# Autodesk Inventor assembly: VER2.0_MIR_CPY_MIR1
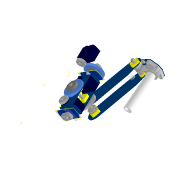
[picture p0: Inventor's stored thumbnail of the model, 180x180]
Saved by Autodesk Inventor 2020.5 (Build 245400000, 400)
## iProperties
Created: 2022-10-31
Part Number: VER2.0_MIR_CPY_MIR1
Document SubType Name: Assembly
Designer: Administrator
Author: Administrator
## Documents named in this file (17)
- C:\Users\Administrator\Documents\kamuy2\kamuy2\VER2.0_MIR_CPY_MIR1.iam
- C:\Users\Administrator\Documents\kamuy2\kamuy2\Parts\Part2_MIR_CPY_MIR1.ipt
- C:\Users\Administrator\Documents\kamuy2\kamuy2\Parts\x-540_idle_MIR_CPY_MIR1.ipt
- C:\Users\Administrator\Documents\kamuy2\kamuy2\Parts\GEABP1.0-32-10-A-12-KFC22-K3_Autodesk_Inventor_2020_20221101\AIS2020\GEABP1_0-32-10-A-12-KFC22-K3_MIR_CPY_MIR1.iam
- C:\Users\Administrator\Documents\kamuy2\kamuy2\Parts\GEYK1.0-70-10-B-10K_Autodesk_Inventor_2020_20221114\AIS2020\GEYK1_0-70-10-B-10K_MIR_CPY_MIR1.iam
- C:\Users\Administrator\Documents\kamuy2\kamuy2\Part16_MIR_CPY_MIR1.ipt
- C:\Users\Administrator\Documents\kamuy2\kamuy2\Part1_MIR_CPY_MIR1.ipt
- C:\Users\Administrator\Documents\kamuy2\kamuy2\Part13_MIR_CPY_MIR1.ipt
- C:\Users\Administrator\Documents\kamuy2\kamuy2\Part17_MIR_CPY_MIR1.ipt
- C:\Users\Administrator\Documents\kamuy2\kamuy2\Parts\SMYHF10_STEP_AP203AP214\SMYHF10_203_MIR_CPY_MIR1.ipt
- C:\Users\Administrator\Documents\kamuy2\kamuy2\Parts\BGHK6800VV-30_Autodesk_Inventor_2020_20221102\AIS2020\BGHK6800VV-30_MIR_CPY_MIR1.iam
- C:\Users\Administrator\Documents\kamuy2\kamuy2\Parts\XW540.N105.I101_MIR_CPY_MIR1.ipt
- C:\Users\Administrator\Documents\kamuy2\kamuy2\Parts\NSFMKR10-67-KA22-A20_Autodesk_Inventor_2020_20221116\AIS2020\NSFMKR10-67-KA22-A20_MIR_CPY_MIR1.iam
- C:\Users\Administrator\Documents\kamuy2\kamuy2\Parts\NSFMR10-37_Autodesk_Inventor_2020_20221116\AIS2020\NSFMR10-37(000_000)_MIR_CPY_MIR1.iam
- C:\Users\Administrator\Documents\kamuy2\kamuy2\Parts\NSFMKRRA10-144-F3-S6-KA5-A18-KB108.5-B11_Autodesk_Inventor_2020_20221117\AIS2020\NSFMKRRA10-144-F3-S6-KA5-A18-KB108_5-B11_MIR_CPY_MIR1.iam
- C:\Users\Administrator\Documents\kamuy2\kamuy2\LEG_MIR_MIR2.iam
- C:\Users\Administrator\Documents\kamuy2\kamuy2\Parts\BGTAB6900VV_Autodesk_Inventor_2020_20221121\AIS2020\BGTAB6900VV_MIR.iam
## Components (26 placed, 16 different names)
1. Part2_MIR_CPY_MIR1:1
2. x-540_idle_MIR_CPY_MIR1:1 — メイト:51, メイト:50, フラッシュ:68, フラッシュ:66, フラッシュ:58, メイト:258, メイト:154, メイト:166, フラッシュ:103, メイト:256
3. GEABP1_0-32-10-A-12-KFC22-K3_MIR_CPY_MIR1:1 [sub-assembly] — メイト:51, メイト:50, フラッシュ:31
4. GEYK1_0-70-10-B-10K_MIR_CPY_MIR1:1 [sub-assembly] — フラッシュ:61, フラッシュ:136, メイト:248
5. x-540_idle_MIR_CPY_MIR1:2 — フラッシュ:68, フラッシュ:66, フラッシュ:58, メイト:86, メイト:85, メイト:168, フラッシュ:100, メイト:183, メイト:180, メイト:179, メイト:178
6. GEABP1_0-32-10-A-12-KFC22-K3_MIR_CPY_MIR1:2 [sub-assembly] — フラッシュ:61, メイト:86, メイト:85
7. Part16_MIR_CPY_MIR1:1 — メイト:258, フラッシュ:92, メイト:170
8. Part16_MIR_CPY_MIR1:2 — メイト:168, メイト:154, フラッシュ:92, メイト:66, フラッシュ:141, メイト:67
9. Part1_MIR_CPY_MIR1:1 — メイト:66, フラッシュ:141, フラッシュ:100
10. Part1_MIR_CPY_MIR1:2 — メイト:183, メイト:170, メイト:166
11. Part13_MIR_CPY_MIR1:1 — フラッシュ:103, フラッシュ:108, フラッシュ:104, メイト:172, メイト:208
12. Part17_MIR_CPY_MIR1:1 — フラッシュ:108, フラッシュ:104, メイト:172, フラッシュ:105, メイト:174, メイト:177
13. SMYHF10_203_MIR_CPY_MIR1:1 — フラッシュ:105, メイト:174, メイト:254
14. GEYK1_0-70-10-B-10K_MIR_CPY_MIR1:2 [sub-assembly] — メイト:177, メイト:207, メイト:42
15. Part13_MIR_CPY_MIR1:2 — メイト:180, メイト:179, メイト:178, フラッシュ:110, メイト:194, メイト:214
16. SMYHF10_203_MIR_CPY_MIR1:2 — メイト:187, メイト:185, メイト:213
17. Part17_MIR_CPY_MIR1:2 — フラッシュ:110, メイト:194, メイト:187, メイト:185, メイト:211, メイト:215, メイト:69
18. GEABP1_0-32-10-A-12-KFC22-K3_MIR_CPY_MIR1:3 [sub-assembly] — メイト:204, メイト:203
19. XW540.N105.I101_MIR_CPY_MIR1:1 — メイト:204, メイト:203, メイト:41
20. NSFMKR10-67-KA22-A20_MIR_CPY_MIR1:1 [sub-assembly] — メイト:254, メイト:208, メイト:207, メイト:40
21. BGHK6800VV-30_MIR_CPY_MIR1:2 [sub-assembly] — メイト:211, メイト:212
22. NSFMR10-37(000_000)_MIR_CPY_MIR1:1 [sub-assembly] — メイト:215, メイト:214, メイト:213, メイト:212, メイト:68
23. NSFMKRRA10-144-F3-S6-KA5-A18-KB108_5-B11_MIR_CPY_MIR1:1 [sub-assembly] — メイト:67, メイト:256, フラッシュ:136, メイト:248, メイト:64
24. LEG_MIR_MIR2:1 [sub-assembly] — フラッシュ:31, メイト:64
25. BGTAB6900VV_MIR:1 [sub-assembly] — メイト:69, メイト:68, フラッシュ:19
26. BGTAB6900VV_MIR:2 [sub-assembly] — メイト:40, メイト:41, メイト:42, フラッシュ:19
## Relationships (54: Mate 39, Flush 15)
- メイト:51 [Mate]: x-540_idle_MIR_CPY_MIR1:1 ↔ GEABP1_0-32-10-A-12-KFC22-K3_MIR_CPY_MIR1:1
- メイト:50 [Mate] (4 mm): x-540_idle_MIR_CPY_MIR1:1 ↔ GEABP1_0-32-10-A-12-KFC22-K3_MIR_CPY_MIR1:1
- フラッシュ:68 [Flush]: x-540_idle_MIR_CPY_MIR1:1 ↔ x-540_idle_MIR_CPY_MIR1:2
- フラッシュ:66 [Flush]: x-540_idle_MIR_CPY_MIR1:1 ↔ x-540_idle_MIR_CPY_MIR1:2
- フラッシュ:58 [Flush]: x-540_idle_MIR_CPY_MIR1:1 ↔ x-540_idle_MIR_CPY_MIR1:2
- フラッシュ:61 [Flush]: GEYK1_0-70-10-B-10K_MIR_CPY_MIR1:1 ↔ GEABP1_0-32-10-A-12-KFC22-K3_MIR_CPY_MIR1:2
- メイト:86 [Mate] (4 mm): x-540_idle_MIR_CPY_MIR1:2 ↔ GEABP1_0-32-10-A-12-KFC22-K3_MIR_CPY_MIR1:2
- メイト:85 [Mate]: x-540_idle_MIR_CPY_MIR1:2 ↔ GEABP1_0-32-10-A-12-KFC22-K3_MIR_CPY_MIR1:2
- メイト:258 [Mate] (15.591 mm): x-540_idle_MIR_CPY_MIR1:1 ↔ Part16_MIR_CPY_MIR1:1
- メイト:168 [Mate] (15.591 mm): x-540_idle_MIR_CPY_MIR1:2 ↔ Part16_MIR_CPY_MIR1:2
- メイト:154 [Mate] (15.591 mm): x-540_idle_MIR_CPY_MIR1:1 ↔ Part16_MIR_CPY_MIR1:2
- フラッシュ:92 [Flush]: Part16_MIR_CPY_MIR1:1 ↔ Part16_MIR_CPY_MIR1:2
- メイト:66 [Mate]: Part16_MIR_CPY_MIR1:2 ↔ Part1_MIR_CPY_MIR1:1
- フラッシュ:141 [Flush] (12.859 mm): Part16_MIR_CPY_MIR1:2 ↔ Part1_MIR_CPY_MIR1:1
- フラッシュ:100 [Flush]: x-540_idle_MIR_CPY_MIR1:2 ↔ Part1_MIR_CPY_MIR1:1
- メイト:183 [Mate]: x-540_idle_MIR_CPY_MIR1:2 ↔ Part1_MIR_CPY_MIR1:2
- メイト:170 [Mate]: Part16_MIR_CPY_MIR1:1 ↔ Part1_MIR_CPY_MIR1:2
- メイト:166 [Mate]: x-540_idle_MIR_CPY_MIR1:1 ↔ Part1_MIR_CPY_MIR1:2
- フラッシュ:103 [Flush]: x-540_idle_MIR_CPY_MIR1:1 ↔ Part13_MIR_CPY_MIR1:1
- フラッシュ:108 [Flush]: Part13_MIR_CPY_MIR1:1 ↔ Part17_MIR_CPY_MIR1:1
- フラッシュ:104 [Flush]: Part13_MIR_CPY_MIR1:1 ↔ Part17_MIR_CPY_MIR1:1
- メイト:172 [Mate] (15 mm): Part13_MIR_CPY_MIR1:1 ↔ Part17_MIR_CPY_MIR1:1
- フラッシュ:105 [Flush] (0.1 mm): Part17_MIR_CPY_MIR1:1 ↔ SMYHF10_203_MIR_CPY_MIR1:1
- メイト:174 [Mate]: Part17_MIR_CPY_MIR1:1 ↔ SMYHF10_203_MIR_CPY_MIR1:1
- メイト:177 [Mate] (5 mm): Part17_MIR_CPY_MIR1:1 ↔ GEYK1_0-70-10-B-10K_MIR_CPY_MIR1:2
- メイト:180 [Mate]: x-540_idle_MIR_CPY_MIR1:2 ↔ Part13_MIR_CPY_MIR1:2
- メイト:179 [Mate]: x-540_idle_MIR_CPY_MIR1:2 ↔ Part13_MIR_CPY_MIR1:2
- メイト:178 [Mate]: x-540_idle_MIR_CPY_MIR1:2 ↔ Part13_MIR_CPY_MIR1:2
- フラッシュ:110 [Flush]: Part13_MIR_CPY_MIR1:2 ↔ Part17_MIR_CPY_MIR1:2
- メイト:194 [Mate] (15 mm): Part13_MIR_CPY_MIR1:2 ↔ Part17_MIR_CPY_MIR1:2
- メイト:187 [Mate]: SMYHF10_203_MIR_CPY_MIR1:2 ↔ Part17_MIR_CPY_MIR1:2
- メイト:185 [Mate]: SMYHF10_203_MIR_CPY_MIR1:2 ↔ Part17_MIR_CPY_MIR1:2
- メイト:204 [Mate]: GEABP1_0-32-10-A-12-KFC22-K3_MIR_CPY_MIR1:3 ↔ XW540.N105.I101_MIR_CPY_MIR1:1
- メイト:203 [Mate]: GEABP1_0-32-10-A-12-KFC22-K3_MIR_CPY_MIR1:3 ↔ XW540.N105.I101_MIR_CPY_MIR1:1
- メイト:254 [Mate]: SMYHF10_203_MIR_CPY_MIR1:1 ↔ NSFMKR10-67-KA22-A20_MIR_CPY_MIR1:1
- メイト:208 [Mate]: Part13_MIR_CPY_MIR1:1 ↔ NSFMKR10-67-KA22-A20_MIR_CPY_MIR1:1
- メイト:207 [Mate]: GEYK1_0-70-10-B-10K_MIR_CPY_MIR1:2 ↔ NSFMKR10-67-KA22-A20_MIR_CPY_MIR1:1
- メイト:211 [Mate] (4 mm): Part17_MIR_CPY_MIR1:2 ↔ BGHK6800VV-30_MIR_CPY_MIR1:2
- メイト:215 [Mate]: Part17_MIR_CPY_MIR1:2 ↔ NSFMR10-37(000_000)_MIR_CPY_MIR1:1
- メイト:214 [Mate]: Part13_MIR_CPY_MIR1:2 ↔ NSFMR10-37(000_000)_MIR_CPY_MIR1:1
- メイト:213 [Mate]: SMYHF10_203_MIR_CPY_MIR1:2 ↔ NSFMR10-37(000_000)_MIR_CPY_MIR1:1
- メイト:212 [Mate]: BGHK6800VV-30_MIR_CPY_MIR1:2 ↔ NSFMR10-37(000_000)_MIR_CPY_MIR1:1
- メイト:67 [Mate]: Part16_MIR_CPY_MIR1:2 ↔ NSFMKRRA10-144-F3-S6-KA5-A18-KB108_5-B11_MIR_CPY_MIR1:1
- メイト:256 [Mate] (31.591 mm): x-540_idle_MIR_CPY_MIR1:1 ↔ NSFMKRRA10-144-F3-S6-KA5-A18-KB108_5-B11_MIR_CPY_MIR1:1
- フラッシュ:136 [Flush] (-3 mm): GEYK1_0-70-10-B-10K_MIR_CPY_MIR1:1 ↔ NSFMKRRA10-144-F3-S6-KA5-A18-KB108_5-B11_MIR_CPY_MIR1:1
- メイト:248 [Mate]: GEYK1_0-70-10-B-10K_MIR_CPY_MIR1:1 ↔ NSFMKRRA10-144-F3-S6-KA5-A18-KB108_5-B11_MIR_CPY_MIR1:1
- フラッシュ:31 [Flush]: GEABP1_0-32-10-A-12-KFC22-K3_MIR_CPY_MIR1:1 ↔ LEG_MIR_MIR2:1
- メイト:64 [Mate]: NSFMKRRA10-144-F3-S6-KA5-A18-KB108_5-B11_MIR_CPY_MIR1:1 ↔ LEG_MIR_MIR2:1
- メイト:69 [Mate] (4 mm): Part17_MIR_CPY_MIR1:2 ↔ BGTAB6900VV_MIR:1
- メイト:68 [Mate]: NSFMR10-37(000_000)_MIR_CPY_MIR1:1 ↔ BGTAB6900VV_MIR:1
- メイト:40 [Mate]: NSFMKR10-67-KA22-A20_MIR_CPY_MIR1:1 ↔ BGTAB6900VV_MIR:2
- メイト:41 [Mate] (18.591 mm): XW540.N105.I101_MIR_CPY_MIR1:1 ↔ BGTAB6900VV_MIR:2
- メイト:42 [Mate] (4 mm): GEYK1_0-70-10-B-10K_MIR_CPY_MIR1:2 ↔ BGTAB6900VV_MIR:2
- フラッシュ:19 [Flush]: BGTAB6900VV_MIR:1 ↔ BGTAB6900VV_MIR:2
